# Autodesk Inventor assembly: Base 02
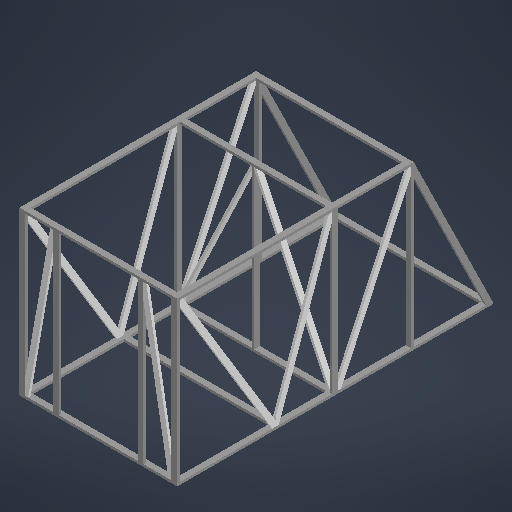
[picture p0: Inventor's stored thumbnail of the model, 512x512]
Saved by Autodesk Inventor 2026 (Build 300175000, 175)
## iProperties
Created: 2024-09-16
Part Number: Base 02
Document SubType Name: Assembly
Designer: User
Author: User
## Documents named in this file (11)
- C:\Users\trott\Documents\UofSC-ASME-Tiger-Burn-Design-2025\CAD\Body\Base 02\Base 02.iam
- C:\Users\trott\Documents\UofSC-ASME-Tiger-Burn-Design-2025\CAD\Body\Base 02\2x4x192.ipt
- C:\Users\trott\Documents\UofSC-ASME-Tiger-Burn-Design-2025\CAD\Body\Base 02\2x4x89.ipt
- C:\Users\trott\Documents\UofSC-ASME-Tiger-Burn-Design-2025\CAD\Body\Base 02\2x4x96.ipt
- C:\Users\trott\Documents\UofSC-ASME-Tiger-Burn-Design-2025\CAD\Body\Base 02\2x4x144.ipt
- C:\Users\trott\Documents\UofSC-ASME-Tiger-Burn-Design-2025\CAD\Body\Base 02\S_2x4x108.675.ipt
- C:\Users\trott\Documents\UofSC-ASME-Tiger-Burn-Design-2025\CAD\Body\Base 02\S_2x4x97.494.ipt
- C:\Users\trott\Documents\UofSC-ASME-Tiger-Burn-Design-2025\CAD\Body\Base 02\S_2x4x106.344.ipt
- C:\Users\trott\Documents\UofSC-ASME-Tiger-Burn-Design-2025\CAD\Body\Base 02\S_2x4x105.918.ipt
- C:\Users\trott\Documents\UofSC-ASME-Tiger-Burn-Design-2025\CAD\Body\Base 02\S_2x4x112.420.ipt
- C:\Users\trott\Documents\UofSC-ASME-Tiger-Burn-Design-2025\CAD\Body\Base 02\S_2x4x101.927.ipt
## Components (32 placed, 10 different names)
1. 2x4x192:1 — Flush:1, Mate:1, Flush:2, Flush:14, Mate:8, Flush:15, Flush:19, Mate:12, Flush:22, Mate:23, Flush:37
2. 2x4x192:2 — Flush:1, Mate:1, Flush:2, Flush:3, Mate:2, Flush:4, Flush:5, Flush:6, Flush:8, Flush:9, Mate:3, Mate:5, Mate:6, Flush:12, Mate:7, Flush:13, Mate:11, Flush:18, Flush:23
3. 2x4x89:1 — Flush:3, Mate:2, Flush:4, Flush:10
4. 2x4x89:2 — Flush:5, Mate:6, Flush:10
5. 2x4x89:3 — Flush:6, Mate:5, Flush:11, Flush:31, Flush:38, Mate:24
6. 2x4x89:5 — Flush:8, Flush:9, Mate:3, Flush:11
7. 2x4x96:1 — Flush:12, Mate:7, Flush:13, Flush:24, Flush:25, Flush:33, Mate:55, Mate:56
8. 2x4x96:2 — Flush:14, Mate:8, Flush:15, Mate:14, Flush:26, Flush:27, Mate:60, Mate:63
9. 2x4x96:5 — Flush:19, Mate:12, Flush:22, Mate:22, Mate:51, Mate:52
10. 2x4x96:6 — Mate:11, Flush:18, Flush:23, Mate:13, Flush:28, Flush:36, Mate:49, Mate:50
11. 2x4x144:1 — Mate:13, Flush:24, Flush:25, Mate:16, Flush:32, Mate:45, Mate:54
12. 2x4x144:2 — Mate:14, Flush:26, Flush:27, Mate:15, Flush:29, Flush:30, Mate:17, Mate:47
13. 2x4x89:6 — Flush:28, Mate:15, Flush:29
14. 2x4x89:7 — Flush:30, Flush:31, Mate:16, Mate:46, Mate:48
15. 2x4x89:8 — Flush:32, Flush:33, Mate:17, Mate:33, Mate:35
16. S_2x4x108.675:1 — Flush:36
17. S_2x4x108.675:2 — Mate:22, Mate:23, Flush:37
18. 2x4x96:9 — Flush:38, Mate:24, Mate:41, Mate:42, Mate:43, Mate:44
19. 2x4x96:10 — Mate:33, Mate:36, Mate:37
20. 2x4x96:11 — Mate:35, Mate:38, Mate:39
21. S_2x4x97.494:1 — Mate:36, Mate:37
22. S_2x4x97.494:2 — Mate:38, Mate:39
23. S_2x4x106.344:1 — Mate:41, Mate:42
24. S_2x4x106.344:2 — Mate:43, Mate:44
25. 2x4x96:14 — Mate:45, Mate:46, Mate:53
26. 2x4x96:15 — Mate:47, Mate:48, Mate:61, Mate:62
27. S_2x4x105.918:1 — Mate:49, Mate:50
28. S_2x4x105.918:2 — Mate:51, Mate:52
29. S_2x4x112.420:1 — Mate:55, Mate:56, Mate:57
30. S_2x4x101.927:1 — Mate:53, Mate:54, Mate:57
31. S_2x4x112.420:2 — Mate:59, Mate:60, Mate:63
32. S_2x4x101.927:2 — Mate:59, Mate:61, Mate:62
## Relationships (77: Mate 46, Flush 31)
- Flush:1: 2x4x192:1 ↔ 2x4x192:2
- Mate:1 (-2438.4 mm): 2x4x192:1 ↔ 2x4x192:2
- Flush:2: 2x4x192:1 ↔ 2x4x192:2
- Flush:3: 2x4x192:2 ↔ 2x4x89:1
- Mate:2: 2x4x192:2 ↔ 2x4x89:1
- Flush:4: 2x4x192:2 ↔ 2x4x89:1
- Flush:5: 2x4x192:2 ↔ 2x4x89:2
- Flush:6: 2x4x192:2 ↔ 2x4x89:3
- Flush:8: 2x4x192:2 ↔ 2x4x89:5
- Flush:9: 2x4x192:2 ↔ 2x4x89:5
- Mate:3: 2x4x192:2 ↔ 2x4x89:5
- Mate:5: 2x4x192:2 ↔ 2x4x89:3
- Mate:6: 2x4x192:2 ↔ 2x4x89:2
- Flush:10 (-1524 mm): 2x4x89:1 ↔ 2x4x89:2
- Flush:11 (-2393.95 mm): 2x4x89:3 ↔ 2x4x89:5
- Flush:12: 2x4x192:2 ↔ 2x4x96:1
- Mate:7: 2x4x192:2 ↔ 2x4x96:1
- Flush:13: 2x4x192:2 ↔ 2x4x96:1
- Flush:14: 2x4x192:1 ↔ 2x4x96:2
- Mate:8: 2x4x192:1 ↔ 2x4x96:2
- Flush:15: 2x4x192:1 ↔ 2x4x96:2
- Mate:11: 2x4x192:2 ↔ 2x4x96:6
- Flush:18: 2x4x192:2 ↔ 2x4x96:6
- Flush:19: 2x4x192:1 ↔ 2x4x96:5
- Mate:12: 2x4x192:1 ↔ 2x4x96:5
- Flush:22 (-1219.2 mm): 2x4x192:1 ↔ 2x4x96:5
- Flush:23 (1219.2 mm): 2x4x192:2 ↔ 2x4x96:6
- Mate:13: 2x4x96:6 ↔ 2x4x144:1
- Flush:24: 2x4x96:1 ↔ 2x4x144:1
- Flush:25: 2x4x96:1 ↔ 2x4x144:1
- Mate:14: 2x4x96:2 ↔ 2x4x144:2
- Flush:26: 2x4x96:2 ↔ 2x4x144:2
- Flush:27: 2x4x96:2 ↔ 2x4x144:2
- Flush:28: 2x4x96:6 ↔ 2x4x89:6
- Mate:15: 2x4x144:2 ↔ 2x4x89:6
- Flush:29: 2x4x144:2 ↔ 2x4x89:6
- Flush:30: 2x4x144:2 ↔ 2x4x89:7
- Flush:31: 2x4x89:3 ↔ 2x4x89:7
- Mate:16: 2x4x144:1 ↔ 2x4x89:7
- Flush:32: 2x4x144:1 ↔ 2x4x89:8
- Flush:33: 2x4x96:1 ↔ 2x4x89:8
- Mate:17: 2x4x144:2 ↔ 2x4x89:8
- Flush:36: 2x4x96:6 ↔ S_2x4x108.675:1
- Mate:22: 2x4x96:5 ↔ S_2x4x108.675:2
- Mate:23: 2x4x192:1 ↔ S_2x4x108.675:2
- Flush:37: 2x4x192:1 ↔ S_2x4x108.675:2
- Flush:38: 2x4x89:3 ↔ 2x4x96:9
- Mate:24: 2x4x89:3 ↔ 2x4x96:9
- Mate:33: 2x4x89:8 ↔ 2x4x96:10
- Mate:35: 2x4x89:8 ↔ 2x4x96:11
- Mate:36: 2x4x96:10 ↔ S_2x4x97.494:1
- Mate:37: 2x4x96:10 ↔ S_2x4x97.494:1
- Mate:38: 2x4x96:11 ↔ S_2x4x97.494:2
- Mate:39: 2x4x96:11 ↔ S_2x4x97.494:2
- Mate:41: 2x4x96:9 ↔ S_2x4x106.344:1
- Mate:42: 2x4x96:9 ↔ S_2x4x106.344:1
- Mate:43: 2x4x96:9 ↔ S_2x4x106.344:2
- Mate:44: 2x4x96:9 ↔ S_2x4x106.344:2
- Mate:45: 2x4x144:1 ↔ 2x4x96:14
- Mate:46: 2x4x89:7 ↔ 2x4x96:14
- Mate:47: 2x4x144:2 ↔ 2x4x96:15
- Mate:48: 2x4x89:7 ↔ 2x4x96:15
- Mate:49: 2x4x96:6 ↔ S_2x4x105.918:1
- Mate:50: 2x4x96:6 ↔ S_2x4x105.918:1
- Mate:51: 2x4x96:5 ↔ S_2x4x105.918:2
- Mate:52: 2x4x96:5 ↔ S_2x4x105.918:2
- Mate:53: 2x4x96:14 ↔ S_2x4x101.927:1
- Mate:54: 2x4x144:1 ↔ S_2x4x101.927:1
- Mate:55: 2x4x96:1 ↔ S_2x4x112.420:1
- Mate:56: 2x4x96:1 ↔ S_2x4x112.420:1
- Mate:57: S_2x4x112.420:1 ↔ S_2x4x101.927:1
- [Mate]: S_2x4x112.420:2 ↔ S_2x4x101.927:2
- Mate:59: S_2x4x112.420:2 ↔ S_2x4x101.927:2
- Mate:60: 2x4x96:2 ↔ S_2x4x112.420:2
- Mate:61: 2x4x96:15 ↔ S_2x4x101.927:2
- Mate:62: 2x4x96:15 ↔ S_2x4x101.927:2
- Mate:63: 2x4x96:2 ↔ S_2x4x112.420:2
## Named parameters: d119_d118 = 0 mm
